# Autodesk Inventor assembly: 조립
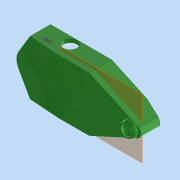
[picture p0: Inventor's stored thumbnail of the model, 180x180]
Saved by Autodesk Inventor 2020 (Build 240168000, 168)
## iProperties
Created: 2020-05-07
Part Number: 조립
Document SubType Name: Assembly
Designer: sbahn
Author: sbahn
## Documents named in this file (5)
- D:\학교 과제\졸업과제\설계\로봇\모델링\조립.iam
- D:\학교 과제\졸업과제\설계\로봇\모델링\본체.ipt
- D:\학교 과제\졸업과제\설계\로봇\모델링\지름 모터 커버.ipt
- D:\학교 과제\졸업과제\설계\로봇\모델링\모터 커버.ipt
- D:\학교 과제\졸업과제\설계\로봇\모델링\전자부품\충방전\충방전.iam
## Components (4 placed, 4 different names)
1. 본체:1 — 플러쉬:1, 플러쉬:2, 플러쉬:3, 메이트:1, 메이트:2, 메이트:3, 메이트:4, 메이트:5, 메이트:6, 메이트:7, 플러쉬:4, 메이트:8
2. 지름 모터 커버:1 — 메이트:1, 메이트:2, 메이트:3
3. 모터 커버:1 — 메이트:4, 메이트:5, 메이트:6
4. 충방전:1 [sub-assembly] — 메이트:7, 플러쉬:4, 메이트:8
## Relationships (12: Mate 8, Flush 4)
- 플러쉬:1 [Flush]: 본체:1
- 플러쉬:2 [Flush]: 본체:1
- 플러쉬:3 [Flush]: 본체:1
- 메이트:1 [Mate]: 본체:1 ↔ 지름 모터 커버:1
- 메이트:2 [Mate]: 본체:1 ↔ 지름 모터 커버:1
- 메이트:3 [Mate]: 본체:1 ↔ 지름 모터 커버:1
- 메이트:4 [Mate]: 본체:1 ↔ 모터 커버:1
- 메이트:5 [Mate]: 본체:1 ↔ 모터 커버:1
- 메이트:6 [Mate]: 본체:1 ↔ 모터 커버:1
- 메이트:7 [Mate]: 본체:1 ↔ 충방전:1
- 플러쉬:4 [Flush]: 본체:1 ↔ 충방전:1
- 메이트:8 [Mate]: 본체:1 ↔ 충방전:1
